# Autodesk Inventor assembly: Опора шаровая 12
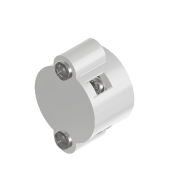
[picture p0: Inventor's stored thumbnail of the model, 180x180]
Saved by Autodesk Inventor 2021.3 (Build 253353010, 353A)
## iProperties
Created: 2021-07-07
Part Number: Опора шаровая 12
Document SubType Name: Assembly
Designer: Михальчик
Author: Михальчик
## Documents named in this file (6)
- C:\Users\Niko\YandexDisk\Гибка Металл\Референсы\шаровая йц\Опора шаровая 12.iam
- C:\Users\Niko\YandexDisk\Гибка Металл\Референсы\шаровая йц\Ш.01.Шарик 12.ipt
- C:\Users\Niko\YandexDisk\Гибка Металл\Референсы\шаровая йц\Ш.02.Шарик 4.ipt
- C:\Users\Niko\YandexDisk\Гибка Металл\Референсы\шаровая йц\Ш.03.Створка.ipt
- C:\Users\Niko\YandexDisk\Гибка Металл\Референсы\шаровая йц\Ш.04.Корпус.ipt
- C:\Users\Niko\Documents\Inventor\Content Center Files\R2021\en-US\ISO 7045(1)\DIN EN ISO 7045 - M2 x 6 - 4.8 - H.ipt
## Components (9 placed, 5 different names)
1. Ш.01.Шарик 12:1 — Mate:1, Tangent:2
2. Ш.03.Створка:1 — Mate:2, Mate:3, Mate:4, Insert:1, Insert:2
3. Ш.04.Корпус:1 — Mate:1, Tangent:1, Mate:2, Mate:3, Mate:4, Mate:5, Mate:6
4. DIN EN ISO 7045 H M2 x 6 - 4.8 - H:1 — Insert:2
5. DIN EN ISO 7045 H M2 x 6 - 4.8 - H:2 — Insert:1
6. Ш.02.Шарик 4:1 — Tangent:1, Tangent:2
7. Ш.02.Шарик 4:2
8. Ш.02.Шарик 4:3
9. Ш.02.Шарик 4:4
## Component patterns: (4 elements, first: Ш.02.Шарик 4:1)
## Relationships (10: Mate 6, Tangent 2, Insert 2)
- Mate:1: Ш.01.Шарик 12:1 ↔ Ш.04.Корпус:1
- Tangent:1: Ш.04.Корпус:1 ↔ Ш.02.Шарик 4:1
- Tangent:2: Ш.01.Шарик 12:1 ↔ Ш.02.Шарик 4:1
- Mate:2: Ш.03.Створка:1 ↔ Ш.04.Корпус:1
- Mate:3: Ш.03.Створка:1 ↔ Ш.04.Корпус:1
- Mate:4: Ш.03.Створка:1 ↔ Ш.04.Корпус:1
- Insert:1: Ш.03.Створка:1 ↔ DIN EN ISO 7045 H M2 x 6 - 4.8 - H:2
- Insert:2: Ш.03.Створка:1 ↔ DIN EN ISO 7045 H M2 x 6 - 4.8 - H:1
- Mate:5: Ш.04.Корпус:1
- Mate:6: Ш.04.Корпус:1
